# Autodesk Inventor assembly: Scoring Platform with Three Sides and Beveled Corners
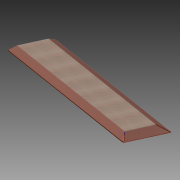
[picture p0: Inventor's stored thumbnail of the model, 180x180]
Saved by Autodesk Inventor 2015 (Build 190159000, 159)
## iProperties
Created: 2015-01-21
Part Number: Scoring Platform with Three Sides and Beveled Corners
Document SubType Name: Assembly
Designer: peters
Author: peters
## Documents named in this file (9)
- C:\Users\peters\Documents\FIRST-Team-1719-CAD-Team\2015 Playing Field\Team 1719 Practice Field\Scoring Platform Version 2 - Construction Design\Scoring Platform with Three Sides and Beveled Corners.iam
- C:\Users\peters\Documents\FIRST-Team-1719-CAD-Team\2015 Playing Field\Team 1719 Practice Field\Scoring Platform Version 2 - Construction Design\Platform - Plywood - 20x72 - 375.ipt
- C:\Users\peters\Documents\FIRST-Team-1719-CAD-Team\2015 Playing Field\Team 1719 Practice Field\Scoring Platform Version 2 - Construction Design\2x4x72.ipt
- C:\Users\peters\Documents\FIRST-Team-1719-CAD-Team\2015 Playing Field\Team 1719 Practice Field\Scoring Platform Version 2 - Construction Design\2x4x13.ipt
- C:\Users\peters\Documents\FIRST-Team-1719-CAD-Team\2015 Playing Field\Team 1719 Practice Field\Scoring Platform Version 2 - Construction Design\Wedge.ipt
- C:\Users\peters\Documents\FIRST-Team-1719-CAD-Team\2015 Playing Field\Team 1719 Practice Field\Scoring Platform Version 2 - Construction Design\Ramp - Side - Trapezoid Assembly.iam
- C:\Users\peters\Documents\FIRST-Team-1719-CAD-Team\2015 Playing Field\Team 1719 Practice Field\Scoring Platform Version 2 - Construction Design\Ramp - End - Trapezoid Assembly.iam
- C:\Users\peters\Documents\FIRST-Team-1719-CAD-Team\2015 Playing Field\Team 1719 Practice Field\Scoring Platform Version 2 - Construction Design\Ramp - Side - Trapezoid Assembly_MIR2.iam
- C:\Users\peters\Documents\FIRST-Team-1719-CAD-Team\2015 Playing Field\Team 1719 Practice Field\Scoring Platform Version 2 - Construction Design\Platform - Polycarbonate - 20x72 - 125.ipt
## Components (22 placed, 8 different names)
1. Platform - Plywood - 20x72 - 375:1 — Mate:3, Mate:4, Flush:1, Flush:2, Flush:3, Flush:4, Mate:5, Mate:6, Flush:5, Flush:6, Flush:21, Flush:22, Flush:23, Mate:24, Mate:40, Flush:26, Flush:27
2. 2x4x72:1 — Mate:3, Flush:3, Flush:4, Mate:7, Mate:13, Mate:14, Mate:15, Mate:16, Flush:11, Flush:12, Flush:13, Flush:14, Flush:16, Flush:18, Mate:22, Flush:24
3. 2x4x72:2 — Mate:4, Flush:1, Flush:2, Mate:8, Mate:9, Mate:10, Mate:11, Mate:12, Flush:7, Flush:8, Flush:9, Flush:10, Flush:15, Flush:17, Mate:36, Mate:37
4. 2x4x13:1 — Mate:6, Flush:6, Mate:7, Mate:39
5. 2x4x13:2 — Mate:5, Flush:5, Mate:8, Mate:21, Flush:19, Flush:20, Flush:25, Mate:38
6. Wedge:1 — Mate:9, Flush:7, Flush:15, Mate:19
7. Wedge:2 — Mate:10, Flush:8, Mate:19
8. Wedge:3 — Mate:11, Flush:9, Mate:20, Mate:23
9. Wedge:4 — Mate:12, Flush:10, Flush:17, Mate:20
10. Wedge:5 — Mate:13, Flush:11, Flush:16, Mate:17
11. Wedge:6 — Mate:14, Flush:12, Mate:17
12. Wedge:7 — Mate:16, Flush:14, Flush:18, Mate:18
13. Wedge:8 — Mate:15, Flush:13, Mate:18
14. Wedge:9 — Mate:21, Flush:19, Flush:22
15. Wedge:10 — Mate:22, Flush:20, Flush:21
16. Ramp - Side - Trapezoid Assembly:1 [sub-assembly] — Mate:23, Flush:23, Mate:24, Mate:25, Mate:26
17. Platform - Plywood - 20x72 - 375:2 — Flush:24, Flush:25, Mate:30, Mate:34, Mate:35
18. Ramp - End - Trapezoid Assembly:1 [sub-assembly] — Mate:30
19. Ramp - Side - Trapezoid Assembly_MIR2:1 [sub-assembly] — Mate:31, Mate:32
20. 2x4x13:3 — Mate:34, Mate:36, Mate:39
21. 2x4x13:4 — Mate:35, Mate:37, Mate:38
22. Platform - Polycarbonate - 20x72 - 125:1 — Mate:40, Flush:26, Flush:27
## Relationships (61: Mate 34, Flush 27)
- Mate:3: Platform - Plywood - 20x72 - 375:1 ↔ 2x4x72:1
- Mate:4: Platform - Plywood - 20x72 - 375:1 ↔ 2x4x72:2
- Flush:1: Platform - Plywood - 20x72 - 375:1 ↔ 2x4x72:2
- Flush:2: Platform - Plywood - 20x72 - 375:1 ↔ 2x4x72:2
- Flush:3: Platform - Plywood - 20x72 - 375:1 ↔ 2x4x72:1
- Flush:4: Platform - Plywood - 20x72 - 375:1 ↔ 2x4x72:1
- Mate:5: Platform - Plywood - 20x72 - 375:1 ↔ 2x4x13:2
- Mate:6: Platform - Plywood - 20x72 - 375:1 ↔ 2x4x13:1
- Flush:5: Platform - Plywood - 20x72 - 375:1 ↔ 2x4x13:2
- Flush:6: Platform - Plywood - 20x72 - 375:1 ↔ 2x4x13:1
- Mate:7: 2x4x72:1 ↔ 2x4x13:1
- Mate:8: 2x4x72:2 ↔ 2x4x13:2
- Mate:9: 2x4x72:2 ↔ Wedge:1
- Mate:10: 2x4x72:2 ↔ Wedge:2
- Mate:11: 2x4x72:2 ↔ Wedge:3
- Mate:12: 2x4x72:2 ↔ Wedge:4
- Mate:13: 2x4x72:1 ↔ Wedge:5
- Mate:14: 2x4x72:1 ↔ Wedge:6
- Mate:15: 2x4x72:1 ↔ Wedge:8
- Mate:16: 2x4x72:1 ↔ Wedge:7
- Flush:7: 2x4x72:2 ↔ Wedge:1
- Flush:8: 2x4x72:2 ↔ Wedge:2
- Flush:9: 2x4x72:2 ↔ Wedge:3
- Flush:10: 2x4x72:2 ↔ Wedge:4
- Flush:11: 2x4x72:1 ↔ Wedge:5
- Flush:12: 2x4x72:1 ↔ Wedge:6
- Flush:13: 2x4x72:1 ↔ Wedge:8
- Flush:14: 2x4x72:1 ↔ Wedge:7
- Flush:15: 2x4x72:2 ↔ Wedge:1
- Flush:16: 2x4x72:1 ↔ Wedge:5
- Flush:17: 2x4x72:2 ↔ Wedge:4
- Flush:18: 2x4x72:1 ↔ Wedge:7
- Mate:17 (491.0667 mm): Wedge:5 ↔ Wedge:6
- Mate:18 (491.0667 mm): Wedge:7 ↔ Wedge:8
- Mate:19 (491.0667 mm): Wedge:1 ↔ Wedge:2
- Mate:20 (491.0667 mm): Wedge:3 ↔ Wedge:4
- Mate:21: 2x4x13:2 ↔ Wedge:9
- Mate:22: 2x4x72:1 ↔ Wedge:10
- Flush:19: 2x4x13:2 ↔ Wedge:9
- Flush:20: 2x4x13:2 ↔ Wedge:10
- Flush:21: Platform - Plywood - 20x72 - 375:1 ↔ Wedge:10
- Flush:22: Platform - Plywood - 20x72 - 375:1 ↔ Wedge:9
- Mate:23: Wedge:3 ↔ Ramp - Side - Trapezoid Assembly:1
- Flush:23: Platform - Plywood - 20x72 - 375:1 ↔ Ramp - Side - Trapezoid Assembly:1
- Mate:24: Platform - Plywood - 20x72 - 375:1 ↔ Ramp - Side - Trapezoid Assembly:1
- Mate:25: Ramp - Side - Trapezoid Assembly:1
- Mate:26: Ramp - Side - Trapezoid Assembly:1
- Flush:24: 2x4x72:1 ↔ Platform - Plywood - 20x72 - 375:2
- Flush:25: 2x4x13:2 ↔ Platform - Plywood - 20x72 - 375:2
- Mate:30: Platform - Plywood - 20x72 - 375:2 ↔ Ramp - End - Trapezoid Assembly:1
- Mate:31: Ramp - Side - Trapezoid Assembly_MIR2:1
- Mate:32: Ramp - Side - Trapezoid Assembly_MIR2:1
- Mate:34: Platform - Plywood - 20x72 - 375:2 ↔ 2x4x13:3
- Mate:35: Platform - Plywood - 20x72 - 375:2 ↔ 2x4x13:4
- Mate:36: 2x4x72:2 ↔ 2x4x13:3
- Mate:37: 2x4x72:2 ↔ 2x4x13:4
- Mate:38 (491.0667 mm): 2x4x13:2 ↔ 2x4x13:4
- Mate:39 (491.0667 mm): 2x4x13:1 ↔ 2x4x13:3
- Mate:40: Platform - Plywood - 20x72 - 375:1 ↔ Platform - Polycarbonate - 20x72 - 125:1
- Flush:26: Platform - Plywood - 20x72 - 375:1 ↔ Platform - Polycarbonate - 20x72 - 125:1
- Flush:27: Platform - Plywood - 20x72 - 375:1 ↔ Platform - Polycarbonate - 20x72 - 125:1
